# Autodesk Inventor assembly: A2017_T2_06
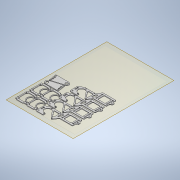
[picture p0: Inventor's stored thumbnail of the model, 180x180]
Saved by Autodesk Inventor 2020 (Build 240168000, 168)
## iProperties
Created: 2021-08-27
Part Number: A2017_T2_06
Document SubType Name: Assembly
Designer: Masato
Author: Masato
## Documents named in this file (5)
- C:\Users\naoki\Documents\Inventor\CitBrains\git_clone\OpenPlatform4_1\コックピット\OpenPlatform_ver3_0\cam\A2017_T2_06.iam
- C:\Users\naoki\Documents\Inventor\CitBrains\git_clone\OpenPlatform4_1\コックピット\OpenPlatform_ver3_0\cam\Disposable_Board.ipt
- C:\Users\naoki\Documents\Inventor\CitBrains\git_clone\OpenPlatform4_1\コックピット\OpenPlatform_ver3_0\LowerBody\Ankle\Ankle_back_frame.ipt
- C:\Users\naoki\Documents\Inventor\CitBrains\git_clone\OpenPlatform4_1\コックピット\OpenPlatform_ver3_0\LowerBody\Ankle\Ankle_side_frame.ipt
- C:\Users\naoki\Documents\Inventor\CitBrains\git_clone\OpenPlatform4_1\コックピット\OpenPlatform_ver3_0\LowerBody\Foot\Foot_front_frame.ipt
## Components (11 placed, 4 different names)
1. Disposable_Board:1 — メイト:2, メイト:1, フラッシュ:1, フラッシュ:2, メイト:4, フラッシュ:3, フラッシュ:4, メイト:5, フラッシュ:5, メイト:7, メイト:8, 正接:1, メイト:11
2. Foot_front_frame:1 — メイト:7, メイト:10, メイト:11
3. Foot_front_frame:2 — メイト:8, 正接:1, メイト:9, メイト:10
4. Ankle_back_frame:1 — メイト:4, フラッシュ:3, フラッシュ:4
5. Ankle_back_frame:2 — メイト:9
6. Ankle_back_frame:3 — メイト:6
7. Ankle_back_frame:4
8. Ankle_side_frame:1 — メイト:5, フラッシュ:5, メイト:6
9. Ankle_side_frame:2
10. Ankle_side_frame:3
11. Ankle_side_frame:4
## Component patterns: (4 elements, first: Ankle_back_frame:1), (4 elements, first: Ankle_side_frame:1)
## Relationships (16: Mate 10, Flush 5, Tangent 1)
- メイト:2 [Mate]: Disposable_Board:1
- メイト:1 [Mate]: Disposable_Board:1
- フラッシュ:1 [Flush]: Disposable_Board:1
- フラッシュ:2 [Flush]: Disposable_Board:1
- メイト:4 [Mate]: Disposable_Board:1 ↔ Ankle_back_frame:1
- フラッシュ:3 [Flush] (2 mm): Disposable_Board:1 ↔ Ankle_back_frame:1
- フラッシュ:4 [Flush] (2 mm): Disposable_Board:1 ↔ Ankle_back_frame:1
- メイト:5 [Mate]: Disposable_Board:1 ↔ Ankle_side_frame:1
- フラッシュ:5 [Flush] (2 mm): Disposable_Board:1 ↔ Ankle_side_frame:1
- メイト:6 [Mate] (2.5 mm): Ankle_back_frame:3 ↔ Ankle_side_frame:1
- メイト:7 [Mate]: Disposable_Board:1 ↔ Foot_front_frame:1
- メイト:8 [Mate]: Disposable_Board:1 ↔ Foot_front_frame:2
- 正接:1 [Tangent] (2 mm): Disposable_Board:1 ↔ Foot_front_frame:2
- メイト:9 [Mate] (2.5 mm): Foot_front_frame:2 ↔ Ankle_back_frame:2
- メイト:10 [Mate] (2.5 mm): Foot_front_frame:1 ↔ Foot_front_frame:2
- メイト:11 [Mate] (-2 mm): Disposable_Board:1 ↔ Foot_front_frame:1
